# Autodesk Inventor assembly: fork_and_mount
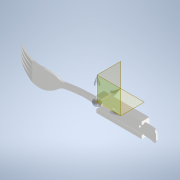
[picture p0: Inventor's stored thumbnail of the model, 180x180]
Saved by Autodesk Inventor 2022 (Build 260153000, 153)
## iProperties
Created: 2022-10-23
Part Number: fork_and_mount
Document SubType Name: Assembly
Designer: Yazawa
Mass: 23.0253 g
Surface Area: 106.018 cm^2
Volume: 13.7015 cm^3
Author: Yazawa
## Documents named in this file (3)
- C:\Users\Yazawa\Documents\GitHub\fork\fork_and_mount.iam
- C:\Users\Yazawa\Documents\GitHub\fork\fork.ipt
- C:\Users\Yazawa\Documents\GitHub\fork\forkmount.ipt
## Components (2 placed, 2 different names)
1. fork:1 — メイト:3, メイト:4, メイト:5
2. forkmount:1 — フラッシュ:1, メイト:1, メイト:2, メイト:3, メイト:4, メイト:5
## Relationships (6: Mate 5, Flush 1)
- フラッシュ:1 [Flush]: forkmount:1
- メイト:1 [Mate]: forkmount:1
- メイト:2 [Mate]: forkmount:1
- メイト:3 [Mate]: fork:1 ↔ forkmount:1
- メイト:4 [Mate]: fork:1 ↔ forkmount:1
- メイト:5 [Mate]: fork:1 ↔ forkmount:1
